# Autodesk Inventor assembly: ведро крутое
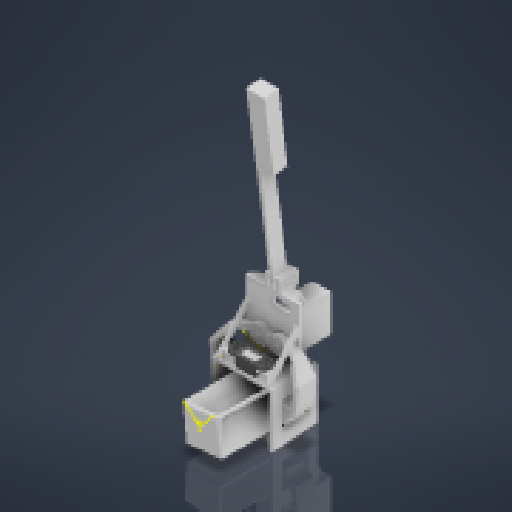
[picture p0: Inventor's stored thumbnail of the model, 512x512]
Saved by Autodesk Inventor 2025 (Build 290162000, 162)
## iProperties
Created: 2025-01-18
Part Number: ведро крутое
Document SubType Name: Assembly
Designer: Phantom
Author: Phantom
## Documents named in this file (8)
- C:\Users\GameHD\Desktop\phantom 16950\ведро крутое.iam
- C:\Users\GameHD\Desktop\phantom 16950\манипулятор 2.ipt
- C:\Users\GameHD\Desktop\phantom 16950\ведро.ipt
- C:\Users\GameHD\Desktop\phantom 16950\ведро 2 гол.ipt
- C:\Users\GameHD\Desktop\phantom 16950\манипулятор 1.ipt
- C:\Users\GameHD\Desktop\phantom 16950\2000-0025-0002\2000-0025-0002.ipt
- C:\Users\GameHD\Desktop\phantom 16950\am-5401 Sample.ipt
- C:\Users\GameHD\Downloads\Telegram Desktop\REV-31-1557\REV-31-1557.ipt
## Components (7 placed, 7 different names)
1. манипулятор 2:1 — Совмещение:3, Совмещение:4
2. ведро:1 — Совмещение:1, Совмещение:2, Заподлицо:1, Совмещение:4, Совмещение:5, Совмещение:6, Совмещение:7, Совмещение:8, Совмещение:9, Совмещение:10
3. ведро 2 гол:1 — Совмещение:6, Совмещение:7
4. манипулятор 1:1 — Совмещение:1, Совмещение:5, Совмещение:8
5. 2000-0025-0002:1 — Совмещение:2, Заподлицо:1, Совмещение:3
6. am-5401 Sample:1
7. REV-31-1557:1 — Совмещение:9, Совмещение:10
## Relationships (11: Mate 10, Flush 1)
- Совмещение:1 [Mate]: ведро:1 ↔ манипулятор 1:1
- Совмещение:2 [Mate]: ведро:1 ↔ 2000-0025-0002:1
- Заподлицо:1 [Flush] (-1 mm): ведро:1 ↔ 2000-0025-0002:1
- Совмещение:3 [Mate]: манипулятор 2:1 ↔ 2000-0025-0002:1
- Совмещение:4 [Mate]: манипулятор 2:1 ↔ ведро:1
- Совмещение:5 [Mate]: ведро:1 ↔ манипулятор 1:1
- Совмещение:6 [Mate]: ведро:1 ↔ ведро 2 гол:1
- Совмещение:7 [Mate]: ведро:1 ↔ ведро 2 гол:1
- Совмещение:8 [Mate]: ведро:1 ↔ манипулятор 1:1
- Совмещение:9 [Mate]: ведро:1 ↔ REV-31-1557:1
- Совмещение:10 [Mate]: ведро:1 ↔ REV-31-1557:1
